# Autodesk Inventor assembly: roller
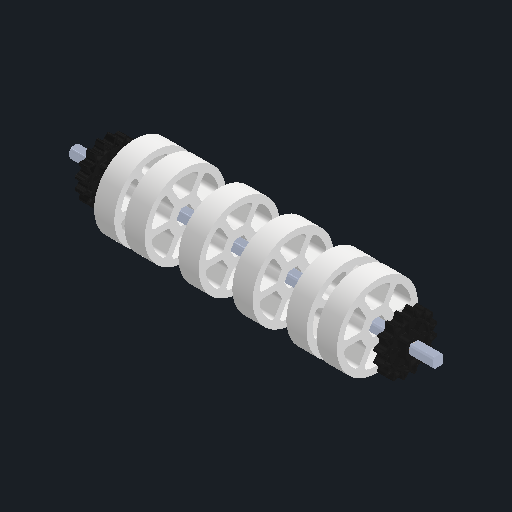
[picture p0: Inventor's stored thumbnail of the model, 512x512]
Saved by Autodesk Inventor 2025 (Build 290162000, 162)
## iProperties
Created: 2024-07-02
Part Number: roller
Document SubType Name: Assembly
Designer: Averey Ku
Author: Averey Ku
## Documents named in this file (7)
- D:\vex_robotics_high_stakes\hardware\cad\EARLY_SEASON\intake\roller.iam
- D:\vex_robotics_high_stakes\hardware\cad\VEX-CAD-Inventor\Motion\Wheels\Flex Wheels\2.000 Flex Wheel\2.000 30A .500.ipt
- D:\vex_robotics_high_stakes\hardware\cad\VEX-CAD-Inventor\Motion\Wheels\Flex Wheels\2.000 Flex Wheel.ipt
- D:\vex_robotics_high_stakes\hardware\cad\VEX-CAD-Inventor\Motion\Shaft HS\Shaft HS\Shaft HS 9.0 in.ipt
- D:\vex_robotics_high_stakes\hardware\cad\VEX-CAD-Inventor\Motion\Shaft HS\Shaft HS.ipt
- D:\vex_robotics_high_stakes\hardware\cad\VEX-CAD-Inventor\Motion\Sprockets\6P Sprocket\6P 16T Sprocket, No Insert.iam
- D:\vex_robotics_high_stakes\hardware\cad\VEX-CAD-Inventor\Motion\Sprockets\6P Sprocket.iam
## Components (9 placed, 3 different names)
1. 2.000 30A .500:1 — Insert:7
2. 2.000 30A .500:2 — Insert:8
3. 2.000 30A .500:3
4. 2.000 30A .500:4
5. 2.000 30A .500:5
6. 2.000 30A .500:6
7. Shaft HS 9.0 in:1
8. 6P 16T Sprocket, No Insert:1 [sub-assembly] — Insert:7
9. 6P 16T Sprocket, No Insert:2 [sub-assembly] — Insert:8
## Relationships (8: Insert 8)
- [Insert] (6.35 mm): 2.000 30A .500:1 ↔ 2.000 30A .500:3
- [Insert] (6.35 mm): 2.000 30A .500:2 ↔ 2.000 30A .500:4
- [Insert] (21.1667 mm): 2.000 30A .500:3 ↔ 2.000 30A .500:5
- [Insert] (21.1667 mm): 2.000 30A .500:4 ↔ 2.000 30A .500:6
- [Insert] (21.1667 mm): 2.000 30A .500:5 ↔ 2.000 30A .500:6
- [Insert] (38.1 mm): 2.000 30A .500:1 ↔ Shaft HS 9.0 in:1
- Insert:7 (11.1125 mm): 2.000 30A .500:1 ↔ 6P 16T Sprocket, No Insert:1
- Insert:8 (11.1125 mm): 2.000 30A .500:2 ↔ 6P 16T Sprocket, No Insert:2
